# Autodesk Inventor assembly: Frame_panels_002
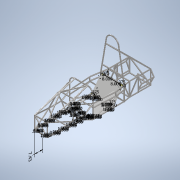
[picture p0: Inventor's stored thumbnail of the model, 180x180]
Saved by Autodesk Inventor 2021 (Build 250183000, 183)
## iProperties
Created: 2020-10-13
Part Number: Frame_panels_002
Document SubType Name: Assembly
Designer: qv17m
_FrameDoc: Frame Assembly
_Version: 25.0.0
Author: qv17m
## Documents named in this file (159)
- C:\Users\mackeycj\Desktop\floorplan2-20201106T152714Z-001\floorplan2\Frame forfloor.iam
- C:\Users\mackeycj\Desktop\floorplan2-20201106T152714Z-001\floorplan2\Skeleton 1602628384448.ipt
- C:\Users\mackeycj\Desktop\floorplan2-20201106T152714Z-001\floorplan2\1602628392525.ipt
- C:\Users\mackeycj\Desktop\floorplan2-20201106T152714Z-001\floorplan2\1602628392562.ipt
- C:\Users\mackeycj\Desktop\floorplan2-20201106T152714Z-001\floorplan2\1602628392597.ipt
- C:\Users\mackeycj\Desktop\floorplan2-20201106T152714Z-001\floorplan2\1602628392633.ipt
- C:\Users\mackeycj\Desktop\floorplan2-20201106T152714Z-001\floorplan2\1602628392669.ipt
- C:\Users\mackeycj\Desktop\floorplan2-20201106T152714Z-001\floorplan2\1602628392753.ipt
- C:\Users\mackeycj\Desktop\floorplan2-20201106T152714Z-001\floorplan2\1602628392788.ipt
- C:\Users\mackeycj\Desktop\floorplan2-20201106T152714Z-001\floorplan2\1602628392824.ipt
- C:\Users\mackeycj\Desktop\floorplan2-20201106T152714Z-001\floorplan2\1602628392859.ipt
- C:\Users\mackeycj\Desktop\floorplan2-20201106T152714Z-001\floorplan2\1602628392894.ipt
- C:\Users\mackeycj\Desktop\floorplan2-20201106T152714Z-001\floorplan2\1602628392929.ipt
- C:\Users\mackeycj\Desktop\floorplan2-20201106T152714Z-001\floorplan2\1602628392967.ipt
- C:\Users\mackeycj\Desktop\floorplan2-20201106T152714Z-001\floorplan2\1602628393002.ipt
- C:\Users\mackeycj\Desktop\floorplan2-20201106T152714Z-001\floorplan2\1602628393084.ipt
- C:\Users\mackeycj\Desktop\floorplan2-20201106T152714Z-001\floorplan2\1602628393120.ipt
- C:\Users\mackeycj\Desktop\floorplan2-20201106T152714Z-001\floorplan2\1602628393155.ipt
- C:\Users\mackeycj\Desktop\floorplan2-20201106T152714Z-001\floorplan2\1602628393192.ipt
- C:\Users\mackeycj\Desktop\floorplan2-20201106T152714Z-001\floorplan2\1602628393227.ipt
- C:\Users\mackeycj\Desktop\floorplan2-20201106T152714Z-001\floorplan2\1602628393262.ipt
- C:\Users\mackeycj\Desktop\floorplan2-20201106T152714Z-001\floorplan2\1602628393297.ipt
- C:\Users\mackeycj\Desktop\floorplan2-20201106T152714Z-001\floorplan2\1602628393332.ipt
- C:\Users\mackeycj\Desktop\floorplan2-20201106T152714Z-001\floorplan2\1602628393380.ipt
- C:\Users\mackeycj\Desktop\floorplan2-20201106T152714Z-001\floorplan2\1602628393415.ipt
- C:\Users\mackeycj\Desktop\floorplan2-20201106T152714Z-001\floorplan2\1602628393451.ipt
- C:\Users\mackeycj\Desktop\floorplan2-20201106T152714Z-001\floorplan2\1602628393487.ipt
- C:\Users\mackeycj\Desktop\floorplan2-20201106T152714Z-001\floorplan2\1602628393522.ipt
- C:\Users\mackeycj\Desktop\floorplan2-20201106T152714Z-001\floorplan2\1602628393556.ipt
- C:\Users\mackeycj\Desktop\floorplan2-20201106T152714Z-001\floorplan2\1602628393591.ipt
- C:\Users\mackeycj\Desktop\floorplan2-20201106T152714Z-001\floorplan2\1602628393626.ipt
- C:\Users\mackeycj\Desktop\floorplan2-20201106T152714Z-001\floorplan2\1602628393661.ipt
- C:\Users\mackeycj\Desktop\floorplan2-20201106T152714Z-001\floorplan2\1602628393741.ipt
- C:\Users\mackeycj\Desktop\floorplan2-20201106T152714Z-001\floorplan2\1602628393777.ipt
- C:\Users\mackeycj\Desktop\floorplan2-20201106T152714Z-001\floorplan2\1602628393812.ipt
- C:\Users\mackeycj\Desktop\floorplan2-20201106T152714Z-001\floorplan2\1602628393848.ipt
- C:\Users\mackeycj\Desktop\floorplan2-20201106T152714Z-001\floorplan2\1602628393883.ipt
- C:\Users\mackeycj\Desktop\floorplan2-20201106T152714Z-001\floorplan2\1602628393919.ipt
- C:\Users\mackeycj\Desktop\floorplan2-20201106T152714Z-001\floorplan2\1602628393955.ipt
- C:\Users\mackeycj\Desktop\floorplan2-20201106T152714Z-001\floorplan2\1602628393991.ipt
- C:\Users\mackeycj\Desktop\floorplan2-20201106T152714Z-001\floorplan2\1602628394070.ipt
- C:\Users\mackeycj\Desktop\floorplan2-20201106T152714Z-001\floorplan2\1602628394106.ipt
- C:\Users\mackeycj\Desktop\floorplan2-20201106T152714Z-001\floorplan2\1602628394141.ipt
- C:\Users\mackeycj\Desktop\floorplan2-20201106T152714Z-001\floorplan2\1602628394177.ipt
- C:\Users\mackeycj\Desktop\floorplan2-20201106T152714Z-001\floorplan2\1602628394212.ipt
- C:\Users\mackeycj\Desktop\floorplan2-20201106T152714Z-001\floorplan2\1602628394247.ipt
- C:\Users\mackeycj\Desktop\floorplan2-20201106T152714Z-001\floorplan2\1602628394281.ipt
- C:\Users\mackeycj\Desktop\floorplan2-20201106T152714Z-001\floorplan2\1602628394316.ipt
- C:\Users\mackeycj\Desktop\floorplan2-20201106T152714Z-001\floorplan2\1602628394394.ipt
- C:\Users\mackeycj\Desktop\floorplan2-20201106T152714Z-001\floorplan2\1602628394431.ipt
- C:\Users\mackeycj\Desktop\floorplan2-20201106T152714Z-001\floorplan2\1602628394467.ipt
- C:\Users\mackeycj\Desktop\floorplan2-20201106T152714Z-001\floorplan2\1602628394503.ipt
- C:\Users\mackeycj\Desktop\floorplan2-20201106T152714Z-001\floorplan2\1602628394538.ipt
- C:\Users\mackeycj\Desktop\floorplan2-20201106T152714Z-001\floorplan2\1602628394574.ipt
- C:\Users\mackeycj\Desktop\floorplan2-20201106T152714Z-001\floorplan2\1602628394610.ipt
- C:\Users\mackeycj\Desktop\floorplan2-20201106T152714Z-001\floorplan2\1602628394646.ipt
- C:\Users\mackeycj\Desktop\floorplan2-20201106T152714Z-001\floorplan2\1602628394723.ipt
- C:\Users\mackeycj\Desktop\floorplan2-20201106T152714Z-001\floorplan2\1602628394759.ipt
- C:\Users\mackeycj\Desktop\floorplan2-20201106T152714Z-001\floorplan2\1602628394795.ipt
- C:\Users\mackeycj\Desktop\floorplan2-20201106T152714Z-001\floorplan2\1602628394830.ipt
- C:\Users\mackeycj\Desktop\floorplan2-20201106T152714Z-001\floorplan2\1602628394864.ipt
- C:\Users\mackeycj\Desktop\floorplan2-20201106T152714Z-001\floorplan2\1602628394899.ipt
- C:\Users\mackeycj\Desktop\floorplan2-20201106T152714Z-001\floorplan2\1602628394970.ipt
- C:\Users\mackeycj\Desktop\floorplan2-20201106T152714Z-001\floorplan2\1602628395020.ipt
- C:\Users\mackeycj\Desktop\floorplan2-20201106T152714Z-001\floorplan2\1602628395056.ipt
- C:\Users\mackeycj\Desktop\floorplan2-20201106T152714Z-001\floorplan2\1602628395092.ipt
- C:\Users\mackeycj\Desktop\floorplan2-20201106T152714Z-001\floorplan2\1602628395127.ipt
- C:\Users\mackeycj\Desktop\floorplan2-20201106T152714Z-001\floorplan2\1602628395162.ipt
- C:\Users\mackeycj\Desktop\floorplan2-20201106T152714Z-001\floorplan2\1602628395198.ipt
- C:\Users\mackeycj\Desktop\floorplan2-20201106T152714Z-001\floorplan2\1602628395234.ipt
- C:\Users\mackeycj\Desktop\floorplan2-20201106T152714Z-001\floorplan2\1602628395269.ipt
- C:\Users\mackeycj\Desktop\floorplan2-20201106T152714Z-001\floorplan2\1602628395305.ipt
- C:\Users\mackeycj\Desktop\floorplan2-20201106T152714Z-001\floorplan2\1602628395381.ipt
- C:\Users\mackeycj\Desktop\floorplan2-20201106T152714Z-001\floorplan2\1602628395416.ipt
- C:\Users\mackeycj\Desktop\floorplan2-20201106T152714Z-001\floorplan2\1602628395451.ipt
- C:\Users\mackeycj\Desktop\floorplan2-20201106T152714Z-001\floorplan2\1602628395487.ipt
- C:\Users\mackeycj\Desktop\floorplan2-20201106T152714Z-001\floorplan2\1602628395523.ipt
- C:\Users\mackeycj\Desktop\floorplan2-20201106T152714Z-001\floorplan2\1602628395559.ipt
- C:\Users\mackeycj\Desktop\floorplan2-20201106T152714Z-001\floorplan2\1602628395594.ipt
- C:\Users\mackeycj\Desktop\floorplan2-20201106T152714Z-001\floorplan2\1602628395630.ipt
- C:\Users\mackeycj\Desktop\floorplan2-20201106T152714Z-001\floorplan2\1602628395706.ipt
- C:\Users\mackeycj\Desktop\floorplan2-20201106T152714Z-001\floorplan2\1602628395742.ipt
- C:\Users\mackeycj\Desktop\floorplan2-20201106T152714Z-001\floorplan2\1602628395778.ipt
- C:\Users\mackeycj\Desktop\floorplan2-20201106T152714Z-001\floorplan2\1602628395813.ipt
- C:\Users\mackeycj\Desktop\floorplan2-20201106T152714Z-001\floorplan2\1602628395849.ipt
- C:\Users\mackeycj\Desktop\floorplan2-20201106T152714Z-001\floorplan2\1602628395884.ipt
- C:\Users\mackeycj\Desktop\floorplan2-20201106T152714Z-001\floorplan2\1602628395955.ipt
- C:\Users\mackeycj\Desktop\floorplan2-20201106T152714Z-001\floorplan2\1602628396034.ipt
- C:\Users\mackeycj\Desktop\floorplan2-20201106T152714Z-001\floorplan2\1602628396069.ipt
- C:\Users\mackeycj\Desktop\floorplan2-20201106T152714Z-001\floorplan2\1602628396105.ipt
- C:\Users\mackeycj\Desktop\floorplan2-20201106T152714Z-001\floorplan2\1602628396140.ipt
- C:\Users\mackeycj\Desktop\floorplan2-20201106T152714Z-001\floorplan2\1602628396176.ipt
- C:\Users\mackeycj\Desktop\floorplan2-20201106T152714Z-001\floorplan2\1602628396212.ipt
- C:\Users\mackeycj\Desktop\floorplan2-20201106T152714Z-001\floorplan2\1602628396247.ipt
- C:\Users\mackeycj\Desktop\floorplan2-20201106T152714Z-001\floorplan2\1602628396283.ipt
- C:\Users\mackeycj\Desktop\floorplan2-20201106T152714Z-001\floorplan2\1602628396360.ipt
- C:\Users\mackeycj\Desktop\floorplan2-20201106T152714Z-001\floorplan2\1602628396396.ipt
- C:\Users\mackeycj\Desktop\floorplan2-20201106T152714Z-001\floorplan2\1602628396431.ipt
- C:\Users\mackeycj\Desktop\floorplan2-20201106T152714Z-001\floorplan2\1602628396466.ipt
- C:\Users\mackeycj\Desktop\floorplan2-20201106T152714Z-001\floorplan2\1602628396501.ipt
- C:\Users\mackeycj\Desktop\floorplan2-20201106T152714Z-001\floorplan2\1602628396537.ipt
- C:\Users\mackeycj\Desktop\floorplan2-20201106T152714Z-001\floorplan2\1602628396574.ipt
- C:\Users\mackeycj\Desktop\floorplan2-20201106T152714Z-001\floorplan2\1602628396609.ipt
- C:\Users\mackeycj\Desktop\floorplan2-20201106T152714Z-001\floorplan2\1602628396656.ipt
- C:\Users\mackeycj\Desktop\floorplan2-20201106T152714Z-001\floorplan2\1602628396691.ipt
- C:\Users\mackeycj\Desktop\floorplan2-20201106T152714Z-001\floorplan2\1602628396726.ipt
- C:\Users\mackeycj\Desktop\floorplan2-20201106T152714Z-001\floorplan2\1602628396762.ipt
- C:\Users\mackeycj\Desktop\floorplan2-20201106T152714Z-001\floorplan2\1602628396797.ipt
- C:\Users\mackeycj\Desktop\floorplan2-20201106T152714Z-001\floorplan2\1602628396832.ipt
- C:\Users\mackeycj\Desktop\floorplan2-20201106T152714Z-001\floorplan2\1602628396868.ipt
- C:\Users\mackeycj\Desktop\floorplan2-20201106T152714Z-001\floorplan2\1602628396904.ipt
- C:\Users\mackeycj\Desktop\floorplan2-20201106T152714Z-001\floorplan2\1602628396939.ipt
- C:\Users\mackeycj\Desktop\floorplan2-20201106T152714Z-001\floorplan2\1602628397017.ipt
- C:\Users\mackeycj\Desktop\floorplan2-20201106T152714Z-001\floorplan2\1602628397052.ipt
- C:\Users\mackeycj\Desktop\floorplan2-20201106T152714Z-001\floorplan2\1602628397088.ipt
- C:\Users\mackeycj\Desktop\floorplan2-20201106T152714Z-001\floorplan2\1602628397123.ipt
- C:\Users\mackeycj\Desktop\floorplan2-20201106T152714Z-001\floorplan2\1602628397158.ipt
- C:\Users\mackeycj\Desktop\floorplan2-20201106T152714Z-001\floorplan2\1602628397194.ipt
- C:\Users\mackeycj\Desktop\floorplan2-20201106T152714Z-001\floorplan2\1602628397229.ipt
- C:\Users\mackeycj\Desktop\floorplan2-20201106T152714Z-001\floorplan2\1602628397264.ipt
- C:\Users\mackeycj\Desktop\floorplan2-20201106T152714Z-001\floorplan2\1602628397343.ipt
- C:\Users\mackeycj\Desktop\floorplan2-20201106T152714Z-001\floorplan2\1602628397378.ipt
- C:\Users\mackeycj\Desktop\floorplan2-20201106T152714Z-001\floorplan2\1602628397413.ipt
- C:\Users\mackeycj\Desktop\floorplan2-20201106T152714Z-001\floorplan2\1602628397449.ipt
- C:\Users\mackeycj\Desktop\floorplan2-20201106T152714Z-001\floorplan2\1602628397484.ipt
- C:\Users\mackeycj\Desktop\floorplan2-20201106T152714Z-001\floorplan2\1602628397519.ipt
- C:\Users\mackeycj\Desktop\floorplan2-20201106T152714Z-001\floorplan2\1602628397555.ipt
- C:\Users\mackeycj\Desktop\floorplan2-20201106T152714Z-001\floorplan2\1602628397590.ipt
- C:\Users\mackeycj\Desktop\floorplan2-20201106T152714Z-001\floorplan2\1602628397666.ipt
- C:\Users\mackeycj\Desktop\floorplan2-20201106T152714Z-001\floorplan2\1602628397701.ipt
- C:\Users\mackeycj\Desktop\floorplan2-20201106T152714Z-001\floorplan2\1602628397737.ipt
- C:\Users\mackeycj\Desktop\floorplan2-20201106T152714Z-001\floorplan2\1602628397772.ipt
- C:\Users\mackeycj\Desktop\floorplan2-20201106T152714Z-001\floorplan2\1602628397807.ipt
- C:\Users\mackeycj\Desktop\floorplan2-20201106T152714Z-001\floorplan2\1602628397843.ipt
- C:\Users\mackeycj\Desktop\floorplan2-20201106T152714Z-001\floorplan2\1602628397879.ipt
- C:\Users\mackeycj\Desktop\floorplan2-20201106T152714Z-001\floorplan2\1602628397914.ipt
- C:\Users\mackeycj\Desktop\floorplan2-20201106T152714Z-001\floorplan2\1602628397991.ipt
- C:\Users\mackeycj\Desktop\floorplan2-20201106T152714Z-001\floorplan2\1602628398027.ipt
- C:\Users\mackeycj\Desktop\floorplan2-20201106T152714Z-001\floorplan2\1602628398062.ipt
- C:\Users\mackeycj\Desktop\floorplan2-20201106T152714Z-001\floorplan2\1602628398098.ipt
- C:\Users\mackeycj\Desktop\floorplan2-20201106T152714Z-001\floorplan2\1602628398133.ipt
- C:\Users\mackeycj\Desktop\floorplan2-20201106T152714Z-001\floorplan2\1602628398168.ipt
- C:\Users\mackeycj\Desktop\floorplan2-20201106T152714Z-001\floorplan2\1602628398203.ipt
- C:\Users\mackeycj\Desktop\floorplan2-20201106T152714Z-001\floorplan2\1602628398239.ipt
- C:\Users\mackeycj\Desktop\floorplan2-20201106T152714Z-001\floorplan2\1602628398282.ipt
- C:\Users\mackeycj\Desktop\floorplan2-20201106T152714Z-001\floorplan2\1602628398317.ipt
- C:\Users\mackeycj\Desktop\floorplan2-20201106T152714Z-001\floorplan2\1602628398353.ipt
- C:\Users\mackeycj\Desktop\floorplan2-20201106T152714Z-001\floorplan2\1602628398388.ipt
- C:\Users\mackeycj\Desktop\floorplan2-20201106T152714Z-001\floorplan2\1602628398423.ipt
- C:\Users\mackeycj\Desktop\floorplan2-20201106T152714Z-001\floorplan2\1602628398459.ipt
- C:\Users\mackeycj\Desktop\floorplan2-20201106T152714Z-001\floorplan2\1602628398494.ipt
- C:\Users\mackeycj\Desktop\floorplan2-20201106T152714Z-001\floorplan2\doorcard2.ipt
- C:\Users\mackeycj\Desktop\floorplan2-20201106T152714Z-001\floorplan2\triangle2.ipt
- C:\Users\mackeycj\Desktop\floorplan2-20201106T152714Z-001\floorplan2\FirewallDiagonal2.ipt
- C:\Users\mackeycj\Desktop\floorplan2-20201106T152714Z-001\floorplan2\firewalltab2.ipt
- C:\Users\mackeycj\Desktop\floorplan2-20201106T152714Z-001\floorplan2\mountingtabsquareshort.ipt
- C:\Users\mackeycj\Desktop\floorplan2-20201106T152714Z-001\floorplan2\floor manufacturing\seatfloorfit.ipt
- C:\Users\mackeycj\Desktop\floorplan2-20201106T152714Z-001\floorplan2\floor manufacturing\frontfloorfit2.ipt
- C:\Users\mackeycj\Desktop\floorplan2-20201106T152714Z-001\floorplan2\floor manufacturing\angledfloorfit2.ipt
## Components (192 placed, 60 different names)
1. Reference Skeleton
2. - 32.794:1
3. - 28.9:1
4. - 21.154:1
5. - 16.083:1
6. - 13:1
7. - 15.5:1
8. - 13:2
9. - 31.689:1
10. - 6.083:1
11. - 13:3
12. - 20:1
13. - 20:2
14. - 28.9:2
15. - 16.083:2
16. - 15.252:1
17. - 14.353:1
18. - 8.09:1
19. - 13:4
20. - 22:1 — Mate:92, Mate:94
21. - 30.454:1
22. - 6.083:2
23. - 20:3
24. - 15.478:1
25. - 20:4
26. - 6.083:3
27. - 6.083:4
28. - 21.154:2
29. - 13:5
30. - 20:5
31. - 23.854:1
32. - 13.5:1
33. - 5.831:1
34. - 20:6
35. - 36.721:1
36. - 1.174:1
37. - 29.4:1 — Mate:44, Mate:45
38. - 13.263:1
39. - 22:2
40. - 0.5:1
41. - 14.353:2
42. - 8.09:2
43. - 13:6
44. - 30.454:2
45. - 16.452:1
46. - 20:7
47. - 13.5:2
48. - 5.831:2
49. - 6.083:5
50. - 6.083:6
51. - 20:8
52. - 15.478:2
53. - 28.9:3
54. - 32.794:2
55. - 16.083:3
56. - 13:7
57. - 13.5:3
58. - 5.831:3
59. - 36.722:1
60. - 11.6:1
61. - 6.708:1
62. - 13.111:1
63. - 20.268:1
64. - 3.5:1
65. - 22.384:1
66. - 10.966:1
67. - 8.322:1
68. - 22:3 — Mate:43, Mate:46, Mate:61, Mate:62, Mate:63, Mate:103, Mate:104, Mate:106
69. - 20:9
70. - 20.268:2
71. - 1.174:2
72. - 29.4:2 — Mate:8, Mate:47
73. - 29.4:3 — Mate:48
74. - 13.263:2
75. - 0.5:2
76. - 1.174:3
77. - 6.708:2
78. - 5.831:4
79. - 13.5:4
80. - 15.5:2
81. - 13:8
82. - 31.689:2
83. - 28.9:4
84. - 16.083:4
85. - 6.708:3
86. - 11.6:2
87. - 11.6:3
88. - 14.461:1
89. - 9.014:1
90. - 6.708:4
91. - 12:1
92. - 11.685:1
93. - 16:1 — Mate:59, Mate:108, Mate:109, Mate:112
94. - 12:2 — Mate:68, Mate:69
95. - 22.384:2
96. - 10.966:2
97. - 8.322:2
98. - 20:10 — Mate:7
99. - 7.854:1
100. - 38.794:1
101. - 14.438:1
102. - 8.09:3
103. - 20.268:3
104. - 1.174:4
105. - 3.5:2
106. - 20.268:4
107. - 6.708:5
108. - 15.252:2
109. - 11.6:4
110. - 4.559:1
111. - 11.685:2
112. - 6.708:6
113. - 20.081:1
114. - 20.081:2
115. - 6.708:7
116. - 12:3 — Mate:32, Mate:70
117. - 16:2
118. - 18.608:1 — Mate:84, Mate:99, Mate:100
119. - 12:4
120. - 11.685:3
121. - 9.014:2
122. - 38.794:2
123. - 7.854:2
124. - 14.438:2
125. - 12:5
126. - 39.56:1
127. - 12:6
128. - 12:7 — Mate:101
129. - 16.971:1
130. - 12:8
131. - 28.188:1
132. - 18.48:1
133. - 8.09:4
134. - 14.461:2
135. - 12:9 — Mate:31, Mate:86
136. - 16.971:2
137. - 6.708:8
138. - 18.608:2 — Mate:71, Mate:72, Mate:95, Mate:96
139. - 20.081:3
140. - 11.685:4
141. - 20.081:4
142. - 4.559:2
143. - 39.56:2
144. - 12:10 — Mate:97
145. - 22:4 — Mate:14, Mate:18, Mate:49, Mate:50
146. - 22:5
147. - 19.571:1
148. - 8:1
149. - 3:3
150. - 3:4
151. doorcard2:1 — Mate:7, Mate:8, Mate:9
152. triangle2:1 — Mate:9
153. FirewallDiagonal2:1 — Mate:16, Mate:19, Mate:89, Mate:90, Mate:91, Mate:93
154. firewalltab2:2 — Mate:14, Mate:16, Mate:90
155. firewalltab2:3 — Mate:18, Mate:19, Mate:89
156. firewalltab2:4 — Mate:91, Mate:92
157. firewalltab2:6 — Mate:93, Mate:94
158. mountingtabsquareshort:1 — Mate:31, Mate:76
159. mountingtabsquareshort:2 — Mate:75, Mate:85, Mate:86
160. mountingtabsquareshort:4 — Mate:32, Mate:78
161. mountingtabsquareshort:5 — Mate:68, Mate:80
162. mountingtabsquareshort:6 — Mate:46, Mate:51
163. mountingtabsquareshort:7 — Mate:43, Mate:52
164. mountingtabsquareshort:8 — Mate:69, Mate:79
165. mountingtabsquareshort:9 — Mate:44
166. seatfloorfit:1 — Mate:51, Mate:52, Mate:53, Mate:54, Mate:55, Mate:57, Mate:88
167. mountingtabsquareshort:10 — Mate:45, Mate:57, Mate:88
168. mountingtabsquareshort:11 — Mate:47, Mate:54
169. mountingtabsquareshort:12 — Mate:48, Mate:53
170. mountingtabsquareshort:13 — Mate:49, Mate:55
171. mountingtabsquareshort:14 — Mate:50
172. frontfloorfit2:1 — Mate:75, Mate:76, Mate:77, Mate:78, Mate:79, Mate:80, Mate:85, Mate:87
173. angledfloorfit2:1 — Mate:64, Mate:65, Mate:66, Mate:67
174. mountingtabsquareshort:15 — Mate:59
175. mountingtabsquareshort:16 — Mate:63, Mate:66
176. mountingtabsquareshort:17 — Mate:62, Mate:65
177. mountingtabsquareshort:18 — Mate:61, Mate:64, Mate:67
178. mountingtabsquareshort:19 — Mate:70, Mate:77
179. mountingtabsquareshort:20 — Mate:72
180. mountingtabsquareshort:21 — Mate:71
181. mountingtabsquareshort:25 — Mate:84
182. mountingtabsquareshort:26 — Mate:87
183. mountingtabsquareshort:27 — Mate:95, Angle:1, Mate:98
184. mountingtabsquareshort:28 — Mate:96, Angle:2, Mate:97, Mate:98
185. mountingtabsquareshort:29 — Mate:99, Mate:102, Angle:3
186. mountingtabsquareshort:30 — Mate:100, Mate:101, Mate:102, Angle:4
187. mountingtabsquareshort:31 — Mate:104, Angle:6, Angle:7, Mate:110, Mate:111
188. mountingtabsquareshort:32 — Mate:108, Mate:114
189. mountingtabsquareshort:33 — Mate:103, Angle:6, Angle:8, Mate:110
190. mountingtabsquareshort:34 — Mate:112, Mate:113, Mate:114
191. mountingtabsquareshort:35 — Mate:109, Mate:113, Angle:9
192. mountingtabsquareshort:36 — Mate:106, Angle:7, Mate:111
## Relationships (79: Mate 71, Angle 8)
- Mate:7: - 20:10 ↔ doorcard2:1
- Mate:8: - 29.4:2 ↔ doorcard2:1
- Mate:9: doorcard2:1 ↔ triangle2:1
- Mate:14: - 22:4 ↔ firewalltab2:2
- Mate:16: FirewallDiagonal2:1 ↔ firewalltab2:2
- Mate:18: - 22:4 ↔ firewalltab2:3
- Mate:19: FirewallDiagonal2:1 ↔ firewalltab2:3
- Mate:31: - 12:9 ↔ mountingtabsquareshort:1
- Mate:32: - 12:3 ↔ mountingtabsquareshort:4
- Mate:43: - 22:3 ↔ mountingtabsquareshort:7
- Mate:44: - 29.4:1 ↔ mountingtabsquareshort:9
- Mate:45: - 29.4:1 ↔ mountingtabsquareshort:10
- Mate:46: - 22:3 ↔ mountingtabsquareshort:6
- Mate:47: - 29.4:2 ↔ mountingtabsquareshort:11
- Mate:48: - 29.4:3 ↔ mountingtabsquareshort:12
- Mate:49: - 22:4 ↔ mountingtabsquareshort:13
- Mate:50: - 22:4 ↔ mountingtabsquareshort:14
- Mate:51: mountingtabsquareshort:6 ↔ seatfloorfit:1
- Mate:52: mountingtabsquareshort:7 ↔ seatfloorfit:1
- Mate:53: seatfloorfit:1 ↔ mountingtabsquareshort:12
- Mate:54: seatfloorfit:1 ↔ mountingtabsquareshort:11
- Mate:55: seatfloorfit:1 ↔ mountingtabsquareshort:13
- Mate:57: seatfloorfit:1 ↔ mountingtabsquareshort:10
- Mate:59: - 16:1 ↔ mountingtabsquareshort:15
- Mate:61: - 22:3 ↔ mountingtabsquareshort:18
- Mate:62: - 22:3 ↔ mountingtabsquareshort:17
- Mate:63: - 22:3 ↔ mountingtabsquareshort:16
- Mate:64: angledfloorfit2:1 ↔ mountingtabsquareshort:18
- Mate:65: angledfloorfit2:1 ↔ mountingtabsquareshort:17
- Mate:66: angledfloorfit2:1 ↔ mountingtabsquareshort:16
- Mate:67: angledfloorfit2:1 ↔ mountingtabsquareshort:18
- Mate:68: - 12:2 ↔ mountingtabsquareshort:5
- Mate:69: - 12:2 ↔ mountingtabsquareshort:8
- Mate:70: - 12:3 ↔ mountingtabsquareshort:19
- Mate:71: - 18.608:2 ↔ mountingtabsquareshort:21
- Mate:72: - 18.608:2 ↔ mountingtabsquareshort:20
- Mate:75: mountingtabsquareshort:2 ↔ frontfloorfit2:1
- Mate:76: mountingtabsquareshort:1 ↔ frontfloorfit2:1
- Mate:77: frontfloorfit2:1 ↔ mountingtabsquareshort:19
- Mate:78: mountingtabsquareshort:4 ↔ frontfloorfit2:1
- Mate:79: mountingtabsquareshort:8 ↔ frontfloorfit2:1
- Mate:80: mountingtabsquareshort:5 ↔ frontfloorfit2:1
- Mate:84: - 18.608:1 ↔ mountingtabsquareshort:25
- Mate:85: mountingtabsquareshort:2 ↔ frontfloorfit2:1
- Mate:86: - 12:9 ↔ mountingtabsquareshort:2
- Mate:87: frontfloorfit2:1 ↔ mountingtabsquareshort:26
- Mate:88: seatfloorfit:1 ↔ mountingtabsquareshort:10
- Mate:89: FirewallDiagonal2:1 ↔ firewalltab2:3
- Mate:90: FirewallDiagonal2:1 ↔ firewalltab2:2
- Mate:91: FirewallDiagonal2:1 ↔ firewalltab2:4
- Mate:92: - 22:1 ↔ firewalltab2:4
- Mate:93: FirewallDiagonal2:1 ↔ firewalltab2:6
- Mate:94: - 22:1 ↔ firewalltab2:6
- Mate:95: - 18.608:2 ↔ mountingtabsquareshort:27
- Angle:1 (0 deg): mountingtabsquareshort:27
- Mate:96: - 18.608:2 ↔ mountingtabsquareshort:28
- Angle:2 (0 deg): mountingtabsquareshort:28
- Mate:97 (177.8 mm): - 12:10 ↔ mountingtabsquareshort:28
- Mate:98 (152.4 mm): mountingtabsquareshort:27 ↔ mountingtabsquareshort:28
- Mate:99: - 18.608:1 ↔ mountingtabsquareshort:29
- Mate:100: - 18.608:1 ↔ mountingtabsquareshort:30
- Mate:101 (177.8 mm): - 12:7 ↔ mountingtabsquareshort:30
- Mate:102 (152.4 mm): mountingtabsquareshort:29 ↔ mountingtabsquareshort:30
- Angle:3 (0 deg): mountingtabsquareshort:29
- Angle:4 (0 deg): mountingtabsquareshort:30
- Mate:103: - 22:3 ↔ mountingtabsquareshort:33
- Mate:104: - 22:3 ↔ mountingtabsquareshort:31
- Mate:106: - 22:3 ↔ mountingtabsquareshort:36
- Angle:6 (0 deg): mountingtabsquareshort:31 ↔ mountingtabsquareshort:33
- Angle:7 (0 deg): mountingtabsquareshort:31 ↔ mountingtabsquareshort:36
- Angle:8 (14 deg): mountingtabsquareshort:33
- Mate:108: - 16:1 ↔ mountingtabsquareshort:32
- Mate:109: - 16:1 ↔ mountingtabsquareshort:35
- Mate:110 (190.5 mm): mountingtabsquareshort:31 ↔ mountingtabsquareshort:33
- Mate:111 (190.5 mm): mountingtabsquareshort:31 ↔ mountingtabsquareshort:36
- Mate:112: - 16:1 ↔ mountingtabsquareshort:34
- Mate:113 (139.7 mm): mountingtabsquareshort:34 ↔ mountingtabsquareshort:35
- Mate:114 (139.7 mm): mountingtabsquareshort:32 ↔ mountingtabsquareshort:34
- Angle:9 (14 deg): mountingtabsquareshort:35
